# Autodesk Inventor assembly: Samenstelling
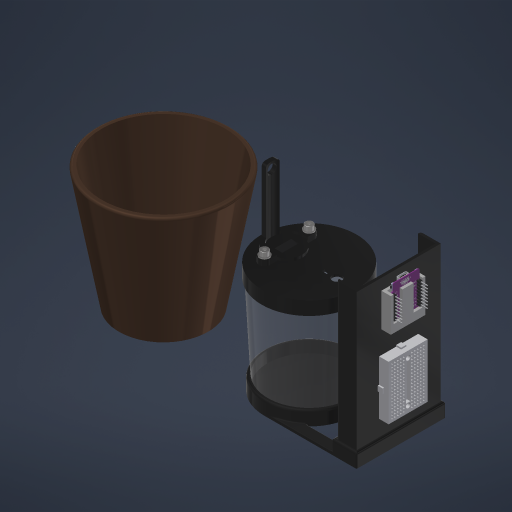
[picture p0: Inventor's stored thumbnail of the model, 512x512]
Saved by Autodesk Inventor 2024 (Build 280153000, 153)
## iProperties
Manager: Bracquené Frank
Company: Hogeschool Gent
Created: 2023-11-03
Part Number: Samenstelling
Catalog Web Link: http://emmausbovenbouw.op-weg.be/
Vendor: Emmaüs Bovenbouw Aalter
Document SubType Name: Assembly
Designer: Louis
Engineer: Declercq St.
Authority: Declercq St.
Title: Wheel of Fortune
Author: Louis
## Documents named in this file (14)
- C:\Autodesk\Vault\Workingfolder - ELM3 - Project IIoT - Plant Irrigation System\Engineering Data\Plant Irrigation System.iam
- C:\Autodesk\Vault\Workingfolder - ELM3 - Project IIoT - Plant Irrigation System\Engineering Data\Base.ipt
- C:\Autodesk\Vault\Workingfolder - ELM3 - Project IIoT - Plant Irrigation System\Engineering Data\Powerbank Holder.ipt
- C:\Autodesk\Vault\Workingfolder - ELM3 - Project IIoT - Plant Irrigation System\Engineering Data\Flowerpot.ipt
- C:\Autodesk\Vault\Workingfolder - ELM3 - Project IIoT - Plant Irrigation System\Engineering Data\Glas - Reservoir.ipt
- C:\Autodesk\Vault\Workingfolder - ELM3 - Project IIoT - Plant Irrigation System\Engineering Data\Reservoir Cap.ipt
- C:\Autodesk\Vault\Workingfolder - ELM3 - Project IIoT - Plant Irrigation System\Engineering Data\Mini breadboard.ipt
- C:\Autodesk\Vault\Workingfolder - ELM3 - Project IIoT - Plant Irrigation System\Engineering Data\LOLIN C3 Mini Holder.ipt
- C:\Autodesk\Vault\Workingfolder - ELM3 - Project IIoT - Plant Irrigation System\Engineering Data\Tube holder.ipt
- C:\Autodesk\Vault\Workingfolder - ELM3 - Project IIoT - Plant Irrigation System\Engineering Data\Filler Cap.ipt
- C:\Autodesk\Vault\Workingfolder - ELM3 - Project IIoT - Plant Irrigation System\Engineering Data\Imported CAD Files\LOLIN C3 Mini\LOLIN C3 Mini.iam
- C:\Autodesk\Vault\Workingfolder - ELM3 - Project IIoT - Plant Irrigation System\Content Center\en-US\DIN 125-1  A\DIN 125 - A 4.3.ipt
- C:\Autodesk\Vault\Workingfolder - ELM3 - Project IIoT - Plant Irrigation System\Content Center\en-US\DIN 912\DIN 912 - M4 x 0.7 x 16 x 14.25.ipt
- C:\Autodesk\Vault\Workingfolder - ELM3 - Project IIoT - Plant Irrigation System\Content Center\en-US\ISO 10511\ISO 10511 - M4.ipt
## Components (18 placed, 13 different names)
1. Base:1 — Mate:1, Mate:2, Mate:3, Flush:1, Mate:4, Mate:5, Mate:6, Mate:9
2. Powerbank Holder:1 — Mate:1, Mate:2, Mate:3, Mate:21, Mate:22, Flush:2, Mate:26, Flush:3
3. Flowerpot:1 — Flush:1, Mate:4
4. Glas - Reservoir:1 — Mate:5, Mate:6, Mate:7, Mate:8
5. Reservoir Cap:1 — Mate:7, Mate:8, Mate:9, Mate:28, Mate:29, Mate:30, Mate:41, Mate:43
6. Mini breadboard:1 — Mate:21, Mate:26, Mate:27
7. LOLIN C3 Mini Holder:1 — Mate:22, Flush:2, Flush:3, Mate:27, Mate:33, Mate:34, Mate:35
8. Tube holder:1 — Mate:28, Mate:29, Mate:30, Mate:31, Mate:32, Mate:36, Mate:37, Mate:38, Mate:39, Mate:40, Mate:42
9. Filler Cap:1 — Mate:31, Mate:32
10. LOLIN C3 Mini:1 [sub-assembly] — Mate:33, Mate:34, Mate:35
11. DIN 125-1 A A 4.3:1 — Mate:36, Mate:37, Insert:1
12. DIN 912 - replaced by DIN EN ISO 4762 M4 x 16:1 — Insert:1
13. DIN 125-1 A A 4.3:2 — Mate:40, Mate:41, Insert:3
14. DIN EN ISO 10511 M4:1 — Insert:3
15. DIN 125-1 A A 4.3:3 — Mate:38, Mate:39, Insert:2
16. DIN 912 - replaced by DIN EN ISO 4762 M4 x 16:2 — Insert:2
17. DIN 125-1 A A 4.3:4 — Mate:42, Mate:43, Insert:4
18. DIN EN ISO 10511 M4:2 — Insert:4
## Relationships (36: Mate 29, Insert 4, Flush 3)
- Mate:1: Base:1 ↔ Powerbank Holder:1
- Mate:2 (0.25 mm): Base:1 ↔ Powerbank Holder:1
- Mate:3 (0.25 mm): Base:1 ↔ Powerbank Holder:1
- Flush:1: Base:1 ↔ Flowerpot:1
- Mate:4: Base:1 ↔ Flowerpot:1
- Mate:5: Base:1 ↔ Glas - Reservoir:1
- Mate:6: Base:1 ↔ Glas - Reservoir:1
- Mate:7: Glas - Reservoir:1 ↔ Reservoir Cap:1
- Mate:8: Glas - Reservoir:1 ↔ Reservoir Cap:1
- Mate:9: Base:1 ↔ Reservoir Cap:1
- Mate:21: Powerbank Holder:1 ↔ Mini breadboard:1
- Mate:22: Powerbank Holder:1 ↔ LOLIN C3 Mini Holder:1
- Flush:2: Powerbank Holder:1 ↔ LOLIN C3 Mini Holder:1
- Mate:26: Powerbank Holder:1 ↔ Mini breadboard:1
- Flush:3 (10 mm): Powerbank Holder:1 ↔ LOLIN C3 Mini Holder:1
- Mate:27 (20 mm): Mini breadboard:1 ↔ LOLIN C3 Mini Holder:1
- Mate:28: Reservoir Cap:1 ↔ Tube holder:1
- Mate:29: Reservoir Cap:1 ↔ Tube holder:1
- Mate:30: Reservoir Cap:1 ↔ Tube holder:1
- Mate:31: Tube holder:1 ↔ Filler Cap:1
- Mate:32: Tube holder:1 ↔ Filler Cap:1
- Mate:33: LOLIN C3 Mini Holder:1 ↔ LOLIN C3 Mini:1
- Mate:34: LOLIN C3 Mini Holder:1 ↔ LOLIN C3 Mini:1
- Mate:35 (0.3 mm): LOLIN C3 Mini Holder:1 ↔ LOLIN C3 Mini:1
- Mate:36: Tube holder:1 ↔ DIN 125-1 A A 4.3:1
- Mate:37: Tube holder:1 ↔ DIN 125-1 A A 4.3:1
- Mate:38: Tube holder:1 ↔ DIN 125-1 A A 4.3:3
- Mate:39: Tube holder:1 ↔ DIN 125-1 A A 4.3:3
- Insert:1: DIN 125-1 A A 4.3:1 ↔ DIN 912 - replaced by DIN EN ISO 4762 M4 x 16:1
- Insert:2: DIN 125-1 A A 4.3:3 ↔ DIN 912 - replaced by DIN EN ISO 4762 M4 x 16:2
- Mate:40: Tube holder:1 ↔ DIN 125-1 A A 4.3:2
- Mate:41: Reservoir Cap:1 ↔ DIN 125-1 A A 4.3:2
- Mate:42: Tube holder:1 ↔ DIN 125-1 A A 4.3:4
- Mate:43: Reservoir Cap:1 ↔ DIN 125-1 A A 4.3:4
- Insert:3: DIN 125-1 A A 4.3:2 ↔ DIN EN ISO 10511 M4:1
- Insert:4: DIN 125-1 A A 4.3:4 ↔ DIN EN ISO 10511 M4:2
